# Autodesk Inventor assembly: 1Ufullsystem
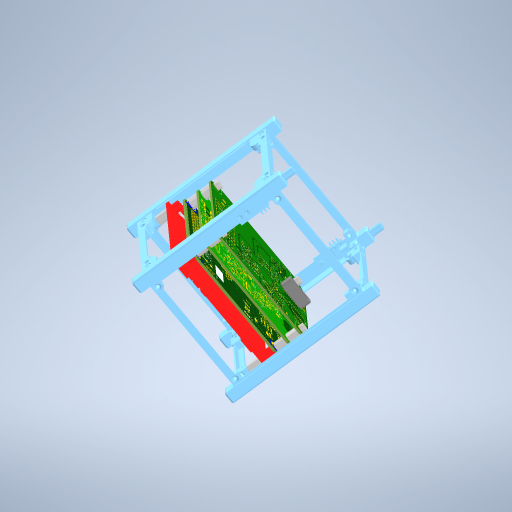
[picture p0: Inventor's stored thumbnail of the model, 512x512]
Saved by Autodesk Inventor 2024 (Build 280153000, 153)
## iProperties
Created: 2023-04-12
Part Number: 1Ufullsystem
Document SubType Name: Assembly
Designer: User
Author: User
## Documents named in this file (10)
- C:\Users\User\Documents\1UFrame\1Ufullsystem.iam
- C:\Users\User\Documents\1UFrame\ISISpace\ISIS CubeSat STS PC104 Skeleton.iam
- C:\Users\User\Documents\1UFrame\PCB_LT_ICR.iam
- C:\Users\User\Documents\1UFrame\PCB_LT_RX-TX.iam
- C:\Users\User\Documents\1UFrame\PCB_LIHU.iam
- C:\Users\User\Documents\1UFrame\PC104_EM-113 Assembly.iam
- C:\Users\User\Downloads\93655A419_Male-Female Threaded Hex Standoff\93655A419_Male-Female Threaded Hex Standoff.ipt
- C:\Users\User\Downloads\93655A704_Male-Female Threaded Hex Standoff (1)\93655A704_Male-Female Threaded Hex Standoff (1).ipt
- C:\Users\User\Downloads\92125A132_18-8 Stainless Steel Hex Drive Flat Head Screw\92125A132_18-8 Stainless Steel Hex Drive Flat Head Screw.ipt
- C:\Users\User\Downloads\91292A112_18-8 Stainless Steel Socket Head Screw\91292A112_18-8 Stainless Steel Socket Head Screw.ipt
## Components (25 placed, 9 different names)
1. ISIS CubeSat STS PC104 Skeleton:1 [sub-assembly] — Mate:117, Mate:118, Mate:119, Mate:120, Mate:121, Mate:122, Mate:123, Mate:124, Mate:128, Mate:129, Mate:130, Mate:131
2. PCB_LT_ICR:1 [sub-assembly] — Mate:82, Mate:83, Mate:86, Mate:87, Mate:90, Mate:91, Mate:93, Mate:94, Mate:132, Mate:133, Mate:134, Mate:135, Mate:136, Mate:137, Mate:138, Mate:139
3. PCB_LT_RX-TX:1 [sub-assembly] — Mate:80, Mate:81, Mate:84, Mate:85, Mate:88, Mate:89, Mate:92, Mate:97, Mate:101, Mate:105, Mate:108
4. PCB_LIHU:2 [sub-assembly] — Mate:95, Mate:99, Mate:100, Mate:103, Mate:104, Mate:106, Mate:107, Mate:109, Mate:110, Mate:111, Mate:112
5. PC104_EM-113 Assembly:1 [sub-assembly] — Mate:109, Mate:110, Mate:111, Mate:112, Mate:113, Mate:114, Mate:115, Mate:116, Mate:125, Mate:126, Mate:127
6. 93655A419_Male-Female Threaded Hex Standoff:1 — Mate:88, Mate:89, Mate:90, Mate:91
7. 93655A419_Male-Female Threaded Hex Standoff:2 — Mate:84, Mate:85, Mate:86, Mate:87, Mate:98
8. 93655A419_Male-Female Threaded Hex Standoff:3 — Mate:92, Mate:93, Mate:94
9. 93655A419_Male-Female Threaded Hex Standoff:4 — Mate:80, Mate:81, Mate:82, Mate:83, Mate:102
10. 93655A419_Male-Female Threaded Hex Standoff:5 — Mate:95, Mate:97, Mate:98, Mate:113
11. 93655A419_Male-Female Threaded Hex Standoff:6 — Mate:99, Mate:100, Mate:101, Mate:102, Mate:115
12. 93655A419_Male-Female Threaded Hex Standoff:7 — Mate:103, Mate:104, Mate:105, Mate:114
13. 93655A419_Male-Female Threaded Hex Standoff:8 — Mate:106, Mate:107, Mate:108, Mate:116
14. 93655A704_Male-Female Threaded Hex Standoff (1):1 — Mate:119, Mate:122, Mate:127
15. 93655A704_Male-Female Threaded Hex Standoff (1):2 — Mate:120, Mate:123, Mate:125, Mate:126
16. 93655A704_Male-Female Threaded Hex Standoff (1):3 — Mate:117, Mate:121
17. 93655A704_Male-Female Threaded Hex Standoff (1):4 — Mate:118, Mate:124
18. 92125A132_18-8 Stainless Steel Hex Drive Flat Head Screw:1 — Mate:130
19. 92125A132_18-8 Stainless Steel Hex Drive Flat Head Screw:2 — Mate:131
20. 92125A132_18-8 Stainless Steel Hex Drive Flat Head Screw:3 — Mate:128
21. 92125A132_18-8 Stainless Steel Hex Drive Flat Head Screw:4 — Mate:129
22. 91292A112_18-8 Stainless Steel Socket Head Screw:1 — Mate:136, Mate:137
23. 91292A112_18-8 Stainless Steel Socket Head Screw:2 — Mate:134, Mate:135
24. 91292A112_18-8 Stainless Steel Socket Head Screw:3 — Mate:138, Mate:139
25. 91292A112_18-8 Stainless Steel Socket Head Screw:4 — Mate:132, Mate:133
## Relationships (59: Mate 59)
- Mate:80: PCB_LT_RX-TX:1 ↔ 93655A419_Male-Female Threaded Hex Standoff:4
- Mate:81: PCB_LT_RX-TX:1 ↔ 93655A419_Male-Female Threaded Hex Standoff:4
- Mate:82: PCB_LT_ICR:1 ↔ 93655A419_Male-Female Threaded Hex Standoff:4
- Mate:83: PCB_LT_ICR:1 ↔ 93655A419_Male-Female Threaded Hex Standoff:4
- Mate:84: PCB_LT_RX-TX:1 ↔ 93655A419_Male-Female Threaded Hex Standoff:2
- Mate:85: PCB_LT_RX-TX:1 ↔ 93655A419_Male-Female Threaded Hex Standoff:2
- Mate:86: PCB_LT_ICR:1 ↔ 93655A419_Male-Female Threaded Hex Standoff:2
- Mate:87: PCB_LT_ICR:1 ↔ 93655A419_Male-Female Threaded Hex Standoff:2
- Mate:88: PCB_LT_RX-TX:1 ↔ 93655A419_Male-Female Threaded Hex Standoff:1
- Mate:89: PCB_LT_RX-TX:1 ↔ 93655A419_Male-Female Threaded Hex Standoff:1
- Mate:90: PCB_LT_ICR:1 ↔ 93655A419_Male-Female Threaded Hex Standoff:1
- Mate:91: PCB_LT_ICR:1 ↔ 93655A419_Male-Female Threaded Hex Standoff:1
- Mate:92: PCB_LT_RX-TX:1 ↔ 93655A419_Male-Female Threaded Hex Standoff:3
- Mate:93: PCB_LT_ICR:1 ↔ 93655A419_Male-Female Threaded Hex Standoff:3
- Mate:94: PCB_LT_ICR:1 ↔ 93655A419_Male-Female Threaded Hex Standoff:3
- Mate:95: PCB_LIHU:2 ↔ 93655A419_Male-Female Threaded Hex Standoff:5
- Mate:97: PCB_LT_RX-TX:1 ↔ 93655A419_Male-Female Threaded Hex Standoff:5
- Mate:98: 93655A419_Male-Female Threaded Hex Standoff:2 ↔ 93655A419_Male-Female Threaded Hex Standoff:5
- Mate:99: PCB_LIHU:2 ↔ 93655A419_Male-Female Threaded Hex Standoff:6
- Mate:100: PCB_LIHU:2 ↔ 93655A419_Male-Female Threaded Hex Standoff:6
- Mate:101: PCB_LT_RX-TX:1 ↔ 93655A419_Male-Female Threaded Hex Standoff:6
- Mate:102: 93655A419_Male-Female Threaded Hex Standoff:4 ↔ 93655A419_Male-Female Threaded Hex Standoff:6
- Mate:103: PCB_LIHU:2 ↔ 93655A419_Male-Female Threaded Hex Standoff:7
- Mate:104: PCB_LIHU:2 ↔ 93655A419_Male-Female Threaded Hex Standoff:7
- Mate:105: PCB_LT_RX-TX:1 ↔ 93655A419_Male-Female Threaded Hex Standoff:7
- Mate:106: PCB_LIHU:2 ↔ 93655A419_Male-Female Threaded Hex Standoff:8
- Mate:107: PCB_LIHU:2 ↔ 93655A419_Male-Female Threaded Hex Standoff:8
- Mate:108: PCB_LT_RX-TX:1 ↔ 93655A419_Male-Female Threaded Hex Standoff:8
- Mate:109: PCB_LIHU:2 ↔ PC104_EM-113 Assembly:1
- Mate:110: PCB_LIHU:2 ↔ PC104_EM-113 Assembly:1
- Mate:111: PCB_LIHU:2 ↔ PC104_EM-113 Assembly:1
- Mate:112: PCB_LIHU:2 ↔ PC104_EM-113 Assembly:1
- Mate:113: PC104_EM-113 Assembly:1 ↔ 93655A419_Male-Female Threaded Hex Standoff:5
- Mate:114: PC104_EM-113 Assembly:1 ↔ 93655A419_Male-Female Threaded Hex Standoff:7
- Mate:115: PC104_EM-113 Assembly:1 ↔ 93655A419_Male-Female Threaded Hex Standoff:6
- Mate:116: PC104_EM-113 Assembly:1 ↔ 93655A419_Male-Female Threaded Hex Standoff:8
- Mate:117: ISIS CubeSat STS PC104 Skeleton:1 ↔ 93655A704_Male-Female Threaded Hex Standoff (1):3
- Mate:118: ISIS CubeSat STS PC104 Skeleton:1 ↔ 93655A704_Male-Female Threaded Hex Standoff (1):4
- Mate:119: ISIS CubeSat STS PC104 Skeleton:1 ↔ 93655A704_Male-Female Threaded Hex Standoff (1):1
- Mate:120: ISIS CubeSat STS PC104 Skeleton:1 ↔ 93655A704_Male-Female Threaded Hex Standoff (1):2
- Mate:121: ISIS CubeSat STS PC104 Skeleton:1 ↔ 93655A704_Male-Female Threaded Hex Standoff (1):3
- Mate:122: ISIS CubeSat STS PC104 Skeleton:1 ↔ 93655A704_Male-Female Threaded Hex Standoff (1):1
- Mate:123: ISIS CubeSat STS PC104 Skeleton:1 ↔ 93655A704_Male-Female Threaded Hex Standoff (1):2
- Mate:124: ISIS CubeSat STS PC104 Skeleton:1 ↔ 93655A704_Male-Female Threaded Hex Standoff (1):4
- Mate:125: PC104_EM-113 Assembly:1 ↔ 93655A704_Male-Female Threaded Hex Standoff (1):2
- Mate:126: PC104_EM-113 Assembly:1 ↔ 93655A704_Male-Female Threaded Hex Standoff (1):2
- Mate:127: PC104_EM-113 Assembly:1 ↔ 93655A704_Male-Female Threaded Hex Standoff (1):1
- Mate:128: ISIS CubeSat STS PC104 Skeleton:1 ↔ 92125A132_18-8 Stainless Steel Hex Drive Flat Head Screw:3
- Mate:129: ISIS CubeSat STS PC104 Skeleton:1 ↔ 92125A132_18-8 Stainless Steel Hex Drive Flat Head Screw:4
- Mate:130: ISIS CubeSat STS PC104 Skeleton:1 ↔ 92125A132_18-8 Stainless Steel Hex Drive Flat Head Screw:1
- Mate:131: ISIS CubeSat STS PC104 Skeleton:1 ↔ 92125A132_18-8 Stainless Steel Hex Drive Flat Head Screw:2
- Mate:132: PCB_LT_ICR:1 ↔ 91292A112_18-8 Stainless Steel Socket Head Screw:4
- Mate:133: PCB_LT_ICR:1 ↔ 91292A112_18-8 Stainless Steel Socket Head Screw:4
- Mate:134: PCB_LT_ICR:1 ↔ 91292A112_18-8 Stainless Steel Socket Head Screw:2
- Mate:135: PCB_LT_ICR:1 ↔ 91292A112_18-8 Stainless Steel Socket Head Screw:2
- Mate:136: PCB_LT_ICR:1 ↔ 91292A112_18-8 Stainless Steel Socket Head Screw:1
- Mate:137: PCB_LT_ICR:1 ↔ 91292A112_18-8 Stainless Steel Socket Head Screw:1
- Mate:138: PCB_LT_ICR:1 ↔ 91292A112_18-8 Stainless Steel Socket Head Screw:3
- Mate:139: PCB_LT_ICR:1 ↔ 91292A112_18-8 Stainless Steel Socket Head Screw:3
